# Autodesk Inventor assembly: Assembly2
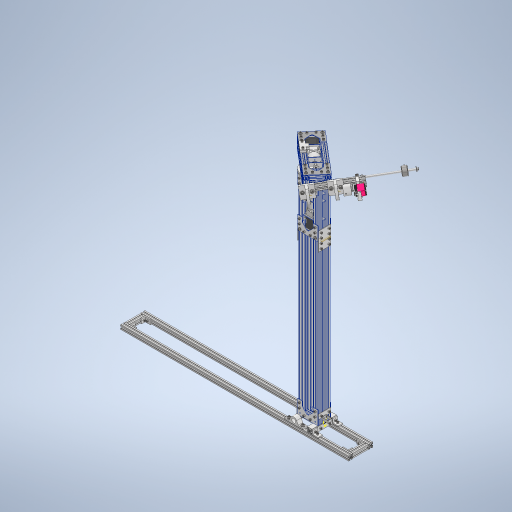
[picture p0: Inventor's stored thumbnail of the model, 512x512]
Saved by Autodesk Inventor 2024 (Build 280153000, 153)
## iProperties
Created: 2025-12-24
Part Number: Assembly2
Document SubType Name: Assembly
Designer: schar
Author: schar
## Documents named in this file (30)
- C:\Users\schar\Desktop\projectBlueprint\AMSTS\hardware\Assembly2.iam
- C:\Users\schar\Desktop\projectBlueprint\AMSTS\hardware\ax4.iam
- C:\Users\schar\Desktop\projectBlueprint\AMSTS\hardware\4ax_plate_joint_asm.iam
- C:\Users\schar\Desktop\projectBlueprint\AMSTS\hardware\ax4_holder_asm.iam
- C:\Users\schar\Desktop\projectBlueprint\AMSTS\hardware\2020_ax_connector_asm.iam
- C:\Users\schar\Desktop\projectBlueprint\AMSTS\hardware\2020_140.ipt
- C:\Users\schar\Desktop\projectBlueprint\AMSTS\hardware\2020_700.ipt
- C:\Users\schar\Desktop\projectBlueprint\AMSTS\hardware\H-Connector_2020-asm.iam
- C:\Users\schar\Desktop\projectBlueprint\AMSTS\hardware\2020_4x2020_ve.ipt
- C:\Users\schar\Desktop\projectBlueprint\AMSTS\hardware\Connect_u2020_asm.iam
- C:\Users\schar\Desktop\projectBlueprint\AMSTS\hardware\4x2020_subaxis-asm.iam
- C:\Users\schar\Desktop\projectBlueprint\AMSTS\hardware\8x7mm_spacer.ipt
- C:\Users\schar\Desktop\projectBlueprint\AMSTS\hardware\608.ipt
- C:\Users\schar\Desktop\projectBlueprint\AMSTS\hardware\base_axis_8mm_2020-asm.iam
- C:\Users\schar\Desktop\projectBlueprint\AMSTS\hardware\8x88_cylinder.ipt
- C:\Users\schar\Desktop\projectBlueprint\AMSTS\hardware\2x2020_hor.ipt
- C:\Users\schar\Desktop\projectBlueprint\AMSTS\hardware\2020_1100.ipt
- C:\Users\schar\Desktop\projectBlueprint\AMSTS\hardware\2020_108.ipt
- C:\Users\schar\Desktop\projectBlueprint\AMSTS\hardware\l-holder_2020-asm.iam
- C:\Users\schar\Desktop\projectBlueprint\AMSTS\hardware\l-holder_2020_spacer.ipt
- C:\Users\schar\Desktop\projectBlueprint\AMSTS\hardware\manual_locker-asm.iam
- C:\Users\schar\Desktop\projectBlueprint\AMSTS\hardware\manual_locker_upper-asm.iam
- C:\Users\schar\Desktop\projectBlueprint\AMSTS\hardware\antenna_holder.iam
- C:\Users\schar\Desktop\projectBlueprint\AMSTS\hardware\gps_holder-asm.iam
- C:\Users\schar\Desktop\projectBlueprint\AMSTS\hardware\servo_holder-asm.iam
- C:\Users\schar\Desktop\projectBlueprint\AMSTS\hardware\DS-3240MG Servo.iam
- C:\Users\schar\Desktop\projectBlueprint\AMSTS\hardware\counterweight-asm.iam
- C:\Users\schar\Desktop\projectBlueprint\AMSTS\hardware\antenna_polarization_rot_conn.ipt
- C:\Users\schar\Documents\Inventor\Content Center Files\R2024\en-US\ISO 4762(1)\DIN EN ISO 4762 - M2 x 16.ipt
- C:\Users\schar\Documents\Inventor\Content Center Files\R2024\en-US\ISO 4762(1)\DIN EN ISO 4762 - M2 x 12.ipt
## Components (49 placed, 29 different names)
1. ax4:1 [sub-assembly] — Angle:1, Tangent:1, Angle:2, Tangent:2, Mate:3, Mate:4, Mate:5, Insert:1, Mate:10, Mate:11, Mate:12, Mate:13, Flush:5, Flush:6, Flush:7, Flush:8, Flush:9, Flush:10, Flush:11, Flush:12, Mate:14, Mate:16
2. 4ax_plate_joint_asm:1 [sub-assembly] — Mate:2, Mate:3, Mate:4
3. ax4_holder_asm:2 [sub-assembly] — Mate:5, Insert:1, Flush:1, Mate:6, Flush:2
4. ax4:2 [sub-assembly] — Flush:1, Mate:6, Flush:2, Mate:7, Mate:8, Mate:75, Flush:51, Mate:76
5. 2020_ax_connector_asm:1 [sub-assembly] — Mate:7, Mate:8, Mate:9, Flush:4, Flush:52
6. 2020_140:1 — Mate:9, Flush:4, Flush:47, Mate:73, Flush:48, Mate:74, Flush:50, Flush:52, Mate:78, Flush:53, Mate:79, Mate:83, Mate:84, Mate:85, Mate:86
7. 2020_700:1 — Mate:11, Flush:11, Flush:12, Flush:14, Flush:17, Mate:19, Flush:21, Flush:37, Flush:45
8. 2020_700:2 — Mate:13, Flush:5, Flush:6, Mate:15, Flush:13, Mate:23, Flush:23, Symmetry:2
9. 2020_700:3 — Mate:10, Flush:9, Flush:10, Mate:17, Flush:15, Mate:18, Flush:16, Flush:20, Mate:71
10. 2020_700:4 — Mate:12, Flush:7, Flush:8, Symmetry:2
11. H-Connector_2020-asm:1 [sub-assembly] — Mate:16, Mate:17, Flush:14
12. H-Connector_2020-asm:2 [sub-assembly] — Mate:14, Mate:15, Flush:13
13. 2020_4x2020_ve:1 — Flush:15, Mate:18, Flush:16, Mate:20, Flush:19
14. 2020_4x2020_ve:2 — Flush:17, Mate:19, Mate:21, Flush:22, Flush:37, Mate:72
15. Connect_u2020_asm:1 [sub-assembly] — Mate:20, Flush:19, Flush:20
16. Connect_u2020_asm:2 [sub-assembly] — Mate:21, Flush:21, Flush:22
17. 4x2020_subaxis-asm:1 [sub-assembly] — Mate:23, Flush:23, Mate:24, Mate:25, Mate:26, Mate:27, Mate:33, Mate:72
18. 8x7mm_spacer:1 — Mate:25, Mate:26, Mate:35
19. 8x7mm_spacer:2 — Mate:24, Mate:27, Cylindrical:1, Mate:34
20. 608:1 — Mate:28, Mate:29, Mate:35
21. 608:2 — Mate:30, Mate:31, Cylindrical:1, Mate:34
22. base_axis_8mm_2020-asm:1 [sub-assembly] — Mate:28, Mate:29, Mate:45, Mate:58
23. base_axis_8mm_2020-asm:2 [sub-assembly] — Mate:30, Mate:31, Mate:44, Flush:29, Flush:38, Mate:62
24. 8x88_cylinder:1 — Mate:33, Mate:41, Mate:58
25. 2020_1100:1 — Mate:43, Flush:26, Flush:27, Mate:45, Mate:46, Mate:47, Flush:40, Mate:66, Mate:99, Mate:105, Flush:59
26. 2020_1100:2 — Flush:24, Mate:42, Flush:25, Mate:44, Flush:29, Mate:61, Flush:39, Mate:64, Mate:101, Flush:55, Mate:102, Flush:56, Flush:57, Mate:106, Flush:58
27. 2x2020_hor:1 — Flush:24, Mate:42, Flush:25, Mate:43, Flush:26, Flush:27, Flush:30, Flush:38, Mate:98, Flush:54, Mate:100
28. 2020_108:1 — Mate:61, Flush:39, Mate:62, Mate:63, Mate:65, Flush:41, Mate:67, Flush:42, Flush:43, Mate:69, Flush:44
29. l-holder_2020-asm:1 [sub-assembly] — Mate:64, Mate:65, Flush:41, Mate:70
30. l-holder_2020-asm:2 [sub-assembly] — Flush:40, Mate:63, Mate:66
31. l-holder_2020_spacer:1 — Mate:67, Flush:42, Flush:43, Flush:46
32. manual_locker-asm:1 [sub-assembly] — Mate:69, Mate:70, Flush:44
33. manual_locker_upper-asm:1 [sub-assembly] — Flush:45, Mate:71, Flush:46
34. antenna_holder:1 [sub-assembly] — Flush:47, Mate:73, Flush:48, Mate:77
35. antenna_holder:2 [sub-assembly] — Mate:74, Flush:50, Mate:77
36. gps_holder-asm:1 [sub-assembly] — Mate:75, Flush:51, Mate:76
37. servo_holder-asm:1 [sub-assembly] — Mate:78, Flush:53, Mate:79, Mate:80, Mate:81, Mate:82
38. DS-3240MG Servo:1 [sub-assembly] — Mate:80, Mate:81, Mate:82, Mate:87, Mate:88, Mate:89
39. counterweight-asm:1 [sub-assembly] — Mate:83, Mate:84, Mate:85, Mate:86
40. antenna_polarization_rot_conn:1 — Mate:87, Mate:88, Mate:89, Mate:90, Mate:91, Mate:92, Mate:93, Mate:94, Mate:95, Mate:96, Mate:97
41. DIN EN ISO 4762 M2 x 16:1 — Mate:91, Mate:92
42. DIN EN ISO 4762 M2 x 16:2 — Mate:90, Mate:93
43. DIN EN ISO 4762 M2 x 12:1 — Mate:94, Mate:96
44. DIN EN ISO 4762 M2 x 12:2 — Mate:95, Mate:97
45. l-holder_2020-asm:3 [sub-assembly] — Mate:98, Mate:99, Flush:54
46. l-holder_2020-asm:4 [sub-assembly] — Mate:100, Mate:101, Flush:55
47. l-holder_2020-asm:5 [sub-assembly] — Mate:104, Mate:105, Flush:59
48. l-holder_2020-asm:6 [sub-assembly] — Mate:103, Mate:106, Flush:58
49. 2x2020_hor:2 — Mate:102, Flush:56, Flush:57, Mate:103, Mate:104
## Relationships (143: Mate 86, Flush 49, Angle 2, Tangent 2, Symmetry 2, Insert 1, CylindricalJoint 1)
- Angle:1 (0 deg): ax4:1
- Tangent:1: ax4:1
- Angle:2 (0 deg): ax4:1
- Tangent:2: ax4:1
- Symmetry:1
- Mate:2: 4ax_plate_joint_asm:1
- Mate:3: ax4:1 ↔ 4ax_plate_joint_asm:1
- Mate:4: ax4:1 ↔ 4ax_plate_joint_asm:1
- Mate:5: ax4:1 ↔ ax4_holder_asm:2
- Insert:1: ax4:1 ↔ ax4_holder_asm:2
- Flush:1: ax4_holder_asm:2 ↔ ax4:2
- Mate:6: ax4_holder_asm:2 ↔ ax4:2
- Flush:2 (-86.8645 mm): ax4_holder_asm:2 ↔ ax4:2
- Mate:7: ax4:2 ↔ 2020_ax_connector_asm:1
- Mate:8: ax4:2 ↔ 2020_ax_connector_asm:1
- Mate:9: 2020_ax_connector_asm:1 ↔ 2020_140:1
- Flush:4: 2020_ax_connector_asm:1 ↔ 2020_140:1
- Mate:10: ax4:1 ↔ 2020_700:3
- Mate:11: ax4:1 ↔ 2020_700:1
- Mate:12: ax4:1 ↔ 2020_700:4
- Mate:13: ax4:1 ↔ 2020_700:2
- Flush:5: ax4:1 ↔ 2020_700:2
- Flush:6: ax4:1 ↔ 2020_700:2
- Flush:7: ax4:1 ↔ 2020_700:4
- Flush:8: ax4:1 ↔ 2020_700:4
- Flush:9: ax4:1 ↔ 2020_700:3
- Flush:10: ax4:1 ↔ 2020_700:3
- Flush:11: ax4:1 ↔ 2020_700:1
- Flush:12: ax4:1 ↔ 2020_700:1
- Mate:14: ax4:1 ↔ H-Connector_2020-asm:2
- Mate:15: 2020_700:2 ↔ H-Connector_2020-asm:2
- Flush:13: 2020_700:2 ↔ H-Connector_2020-asm:2
- Mate:16: ax4:1 ↔ H-Connector_2020-asm:1
- Mate:17: 2020_700:3 ↔ H-Connector_2020-asm:1
- Flush:14: 2020_700:1 ↔ H-Connector_2020-asm:1
- Flush:15: 2020_700:3 ↔ 2020_4x2020_ve:1
- Mate:18: 2020_700:3 ↔ 2020_4x2020_ve:1
- Flush:16: 2020_700:3 ↔ 2020_4x2020_ve:1
- Flush:17: 2020_700:1 ↔ 2020_4x2020_ve:2
- Mate:19: 2020_700:1 ↔ 2020_4x2020_ve:2
- Mate:20: 2020_4x2020_ve:1 ↔ Connect_u2020_asm:1
- Flush:19: 2020_4x2020_ve:1 ↔ Connect_u2020_asm:1
- Flush:20: 2020_700:3 ↔ Connect_u2020_asm:1
- Mate:21: 2020_4x2020_ve:2 ↔ Connect_u2020_asm:2
- Flush:21: 2020_700:1 ↔ Connect_u2020_asm:2
- Flush:22: 2020_4x2020_ve:2 ↔ Connect_u2020_asm:2
- Mate:23: 2020_700:2 ↔ 4x2020_subaxis-asm:1
- Flush:23: 2020_700:2 ↔ 4x2020_subaxis-asm:1
- Mate:24: 4x2020_subaxis-asm:1 ↔ 8x7mm_spacer:2
- Mate:25: 4x2020_subaxis-asm:1 ↔ 8x7mm_spacer:1
- Mate:26: 4x2020_subaxis-asm:1 ↔ 8x7mm_spacer:1
- Mate:27: 4x2020_subaxis-asm:1 ↔ 8x7mm_spacer:2
- Mate:28: 608:1 ↔ base_axis_8mm_2020-asm:1
- Mate:29: 608:1 ↔ base_axis_8mm_2020-asm:1
- Mate:30: 608:2 ↔ base_axis_8mm_2020-asm:2
- Mate:31: 608:2 ↔ base_axis_8mm_2020-asm:2
- Mate:33: 4x2020_subaxis-asm:1 ↔ 8x88_cylinder:1
- Cylindrical:1: 8x7mm_spacer:2 ↔ 608:2
- Mate:34: 8x7mm_spacer:2 ↔ 608:2
- Mate:35: 8x7mm_spacer:1 ↔ 608:1
- Symmetry:2: 2020_700:2 ↔ 2020_700:4
- Mate:41: 8x88_cylinder:1
- Flush:24: 2020_1100:2 ↔ 2x2020_hor:1
- Mate:42: 2020_1100:2 ↔ 2x2020_hor:1
- Flush:25: 2020_1100:2 ↔ 2x2020_hor:1
- Mate:43: 2020_1100:1 ↔ 2x2020_hor:1
- Flush:26: 2020_1100:1 ↔ 2x2020_hor:1
- Flush:27: 2020_1100:1 ↔ 2x2020_hor:1
- Mate:44: base_axis_8mm_2020-asm:2 ↔ 2020_1100:2
- Flush:29: base_axis_8mm_2020-asm:2 ↔ 2020_1100:2
- Mate:45: base_axis_8mm_2020-asm:1 ↔ 2020_1100:1
- Mate:46: 2020_1100:1
- Mate:47: 2020_1100:1
- Flush:30: 2x2020_hor:1
- Mate:58: base_axis_8mm_2020-asm:1 ↔ 8x88_cylinder:1
- Mate:60
- Flush:37: 2020_700:1 ↔ 2020_4x2020_ve:2
- Flush:38 (200 mm): base_axis_8mm_2020-asm:2 ↔ 2x2020_hor:1
- Mate:61: 2020_1100:2 ↔ 2020_108:1
- Flush:39: 2020_1100:2 ↔ 2020_108:1
- Mate:62 (20 mm): base_axis_8mm_2020-asm:2 ↔ 2020_108:1
- Flush:40: 2020_1100:1 ↔ l-holder_2020-asm:2
- Mate:63: 2020_108:1 ↔ l-holder_2020-asm:2
- Mate:64: 2020_1100:2 ↔ l-holder_2020-asm:1
- Mate:65: 2020_108:1 ↔ l-holder_2020-asm:1
- Flush:41: 2020_108:1 ↔ l-holder_2020-asm:1
- Mate:66: 2020_1100:1 ↔ l-holder_2020-asm:2
- Mate:67: 2020_108:1 ↔ l-holder_2020_spacer:1
- Flush:42: 2020_108:1 ↔ l-holder_2020_spacer:1
- Flush:43: 2020_108:1 ↔ l-holder_2020_spacer:1
- Mate:69: 2020_108:1 ↔ manual_locker-asm:1
- Mate:70: l-holder_2020-asm:1 ↔ manual_locker-asm:1
- Flush:44: 2020_108:1 ↔ manual_locker-asm:1
- Flush:45: 2020_700:1 ↔ manual_locker_upper-asm:1
- Mate:71: 2020_700:3 ↔ manual_locker_upper-asm:1
- Flush:46 (-26 mm): l-holder_2020_spacer:1 ↔ manual_locker_upper-asm:1
- Mate:72: 2020_4x2020_ve:2 ↔ 4x2020_subaxis-asm:1
- Flush:47: 2020_140:1 ↔ antenna_holder:1
- Mate:73: 2020_140:1 ↔ antenna_holder:1
- Flush:48 (-19 mm): 2020_140:1 ↔ antenna_holder:1
- Mate:74: 2020_140:1 ↔ antenna_holder:2
- Flush:50 (-19 mm): 2020_140:1 ↔ antenna_holder:2
- Mate:75: ax4:2 ↔ gps_holder-asm:1
- Flush:51: ax4:2 ↔ gps_holder-asm:1
- Mate:76: ax4:2 ↔ gps_holder-asm:1
- Mate:77 (-140 mm): antenna_holder:1 ↔ antenna_holder:2
- Flush:52: 2020_ax_connector_asm:1 ↔ 2020_140:1
- Mate:78: 2020_140:1 ↔ servo_holder-asm:1
- Flush:53: 2020_140:1 ↔ servo_holder-asm:1
- Mate:79: 2020_140:1 ↔ servo_holder-asm:1
- Mate:80: servo_holder-asm:1 ↔ DS-3240MG Servo:1
- Mate:81: servo_holder-asm:1 ↔ DS-3240MG Servo:1
- Mate:82: servo_holder-asm:1 ↔ DS-3240MG Servo:1
- Mate:83: 2020_140:1 ↔ counterweight-asm:1
- Mate:84: 2020_140:1 ↔ counterweight-asm:1
- Mate:85: 2020_140:1 ↔ counterweight-asm:1
- Mate:86 (-40 mm): 2020_140:1 ↔ counterweight-asm:1
- Mate:87: DS-3240MG Servo:1 ↔ antenna_polarization_rot_conn:1
- Mate:88: DS-3240MG Servo:1 ↔ antenna_polarization_rot_conn:1
- Mate:89: DS-3240MG Servo:1 ↔ antenna_polarization_rot_conn:1
- Mate:90: antenna_polarization_rot_conn:1 ↔ DIN EN ISO 4762 M2 x 16:2
- Mate:91: antenna_polarization_rot_conn:1 ↔ DIN EN ISO 4762 M2 x 16:1
- Mate:92: antenna_polarization_rot_conn:1 ↔ DIN EN ISO 4762 M2 x 16:1
- Mate:93: antenna_polarization_rot_conn:1 ↔ DIN EN ISO 4762 M2 x 16:2
- Mate:94: antenna_polarization_rot_conn:1 ↔ DIN EN ISO 4762 M2 x 12:1
- Mate:95: antenna_polarization_rot_conn:1 ↔ DIN EN ISO 4762 M2 x 12:2
- Mate:96: antenna_polarization_rot_conn:1 ↔ DIN EN ISO 4762 M2 x 12:1
- Mate:97: antenna_polarization_rot_conn:1 ↔ DIN EN ISO 4762 M2 x 12:2
- Mate:98: 2x2020_hor:1 ↔ l-holder_2020-asm:3
- Mate:99: 2020_1100:1 ↔ l-holder_2020-asm:3
- Flush:54: 2x2020_hor:1 ↔ l-holder_2020-asm:3
- Mate:100: 2x2020_hor:1 ↔ l-holder_2020-asm:4
- Mate:101: 2020_1100:2 ↔ l-holder_2020-asm:4
- Flush:55: 2020_1100:2 ↔ l-holder_2020-asm:4
- Mate:102: 2020_1100:2 ↔ 2x2020_hor:2
- Flush:56: 2020_1100:2 ↔ 2x2020_hor:2
- Flush:57: 2020_1100:2 ↔ 2x2020_hor:2
- Mate:103: l-holder_2020-asm:6 ↔ 2x2020_hor:2
- Mate:104: l-holder_2020-asm:5 ↔ 2x2020_hor:2
- Mate:105: 2020_1100:1 ↔ l-holder_2020-asm:5
- Mate:106: 2020_1100:2 ↔ l-holder_2020-asm:6
- Flush:58: 2020_1100:2 ↔ l-holder_2020-asm:6
- Flush:59: 2020_1100:1 ↔ l-holder_2020-asm:5
